# Autodesk Inventor assembly: 4-7
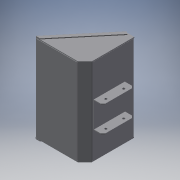
[picture p0: Inventor's stored thumbnail of the model, 180x180]
Saved by Autodesk Inventor 2017 (Build 210142000, 142)
## iProperties
Part Number: 4-7
Material: 一般
Document SubType Name: Assembly
Designer: Brian
Author: Brian
## Documents named in this file (5)
- E:\Brian\檔案\電腦輔助機械設計\PDF2\4-7.iam
- E:\Brian\檔案\電腦輔助機械設計\PDF2\4-4.ipt
- E:\Brian\檔案\電腦輔助機械設計\PDF2\4-5.ipt
- E:\Brian\檔案\電腦輔助機械設計\PDF2\4-6A.ipt
- E:\Brian\檔案\電腦輔助機械設計\PDF2\4-6B.ipt
## Components (4 placed, 4 different names)
1. 4-4:1 — 貼合:2, 貼合:3
2. 4-5:1 — 齊平:1, 貼合:1, 貼合:2, 貼合:3, 貼合:4, 齊平:2, 齊平:3
3. 4-6A:1 — 齊平:1, 貼合:1
4. 4-6B:1 — 貼合:4, 齊平:2, 齊平:3
## Relationships (7: Mate 4, Flush 3)
- 齊平:1 [Flush]: 4-5:1 ↔ 4-6A:1
- 貼合:1 [Mate]: 4-5:1 ↔ 4-6A:1
- 貼合:2 [Mate]: 4-4:1 ↔ 4-5:1
- 貼合:3 [Mate]: 4-4:1 ↔ 4-5:1
- 貼合:4 [Mate]: 4-5:1 ↔ 4-6B:1
- 齊平:2 [Flush]: 4-5:1 ↔ 4-6B:1
- 齊平:3 [Flush]: 4-5:1 ↔ 4-6B:1
